# Autodesk Inventor assembly: finch_ring_straight_fittings
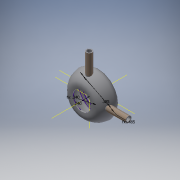
[picture p0: Inventor's stored thumbnail of the model, 180x180]
Saved by Autodesk Inventor 2016 (Build 200138000, 138)
## iProperties
Created: 2016-03-15
Part Number: finch_ring_straight_fittings
Document SubType Name: Assembly
Designer: GentnerLab
Author: GentnerLab
## Documents named in this file (3)
- C:\Users\GentnerLab\Documents\Inventor\Parts\finch_ring_straight_fittings.iam
- C:\Users\GentnerLab\Documents\Inventor\Parts\finch_ring.ipt
- C:\Users\GentnerLab\Documents\Inventor\Parts\straight_fit.ipt
## Components (3 placed, 2 different names)
1. finch_ring:1 — Mate:1, Mate:2
2. straight_fit:1 — Mate:1
3. straight_fit:2 — Mate:2
## Relationships (2: Mate 2)
- Mate:1: finch_ring:1 ↔ straight_fit:1
- Mate:2: finch_ring:1 ↔ straight_fit:2
